# Autodesk Inventor assembly: Camera stage V2 assembly
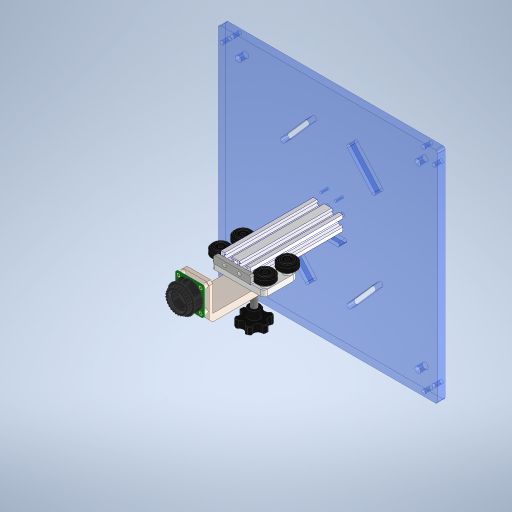
[picture p0: Inventor's stored thumbnail of the model, 512x512]
Saved by Autodesk Inventor 2023 (Build 270158000, 158)
## iProperties
Created: 2020-12-15
Part Number: Camera stage V2 assembly
Document SubType Name: Assembly
Designer: ferrerx
Author: ferrerx
## Documents named in this file (12)
- C:\Users\ferrerx\Desktop\Projects\Prieto-Godino Lab\Drosophila Larvae Behavioural Device\Device design V4\Inventor Assembly\Camera stage V2\Camera stage V2 assembly.iam
- C:\Users\ferrerx\Desktop\Projects\Prieto-Godino Lab\Drosophila Larvae Behavioural Device\Device design V4\Inventor Assembly\cart_spacer.ipt
- C:\Users\ferrerx\Desktop\Projects\Prieto-Godino Lab\Drosophila Larvae Behavioural Device\Device design V4\Inventor Assembly\guide wheel.ipt
- C:\Users\ferrerx\Documents\Inventor\Content Center Files\R2020\en-US\AS 1427(10)\AS 1427 - M5 x 30(7).ipt
- C:\Users\ferrerx\Documents\Inventor\Content Center Files\R2020\en-US\BS 4183(1)\BS 4183 - M5(1).ipt
- C:\Users\ferrerx\Desktop\Projects\Prieto-Godino Lab\Drosophila Larvae Behavioural Device\Device design V4\Inventor Assembly\Camera stage V2\Camera_cart_V2.ipt
- C:\Users\ferrerx\Desktop\Projects\Prieto-Godino Lab\Drosophila Larvae Behavioural Device\Device design V4\Inventor Assembly\Camera stage V2\aluminum profile camera stage.ipt
- C:\Users\ferrerx\Desktop\Projects\Prieto-Godino Lab\Drosophila Larvae Behavioural Device\Device design V4\Inventor Assembly\Camera stage V2\RaspberryPi HQ Camera.ipt
- C:\Users\ferrerx\Desktop\Projects\Prieto-Godino Lab\Drosophila Larvae Behavioural Device\Device design V4\Inventor Assembly\Camera stage V2\Raspberry pi HQ camera holder V2.ipt
- C:\Users\ferrerx\Desktop\Projects\Prieto-Godino Lab\Drosophila Larvae Behavioural Device\Device design V4\Inventor Assembly\Camera stage V2\Z stage Roof V2.ipt
- C:\Users\ferrerx\Desktop\Projects\Prieto-Godino Lab\Drosophila Larvae Behavioural Device\Device design V4\Inventor Assembly\Camera stage V2\Thumb screw.ipt
- C:\Users\ferrerx\Desktop\Projects\Prieto-Godino Lab\Drosophila Larvae Behavioural Device\Device design V4\Inventor Assembly\Camera stage V2\Stop.ipt
## Components (23 placed, 11 different names)
1. cart_spacer:1 — Mate:16, Mate:47, Mate:48, Mate:51
2. cart_spacer:2 — Mate:18, Mate:49, Mate:50, Mate:53
3. cart_spacer:3 — Mate:19, Mate:43, Mate:54
4. cart_spacer:4 — Mate:17, Mate:45, Mate:46, Mate:52
5. guide wheel:1 — Mate:18, Mate:42, Mate:50
6. guide wheel:2 — Mate:17, Mate:40, Mate:46
7. guide wheel:3 — Mate:16, Mate:41, Mate:48
8. guide wheel:4 — Mate:19, Mate:39, Mate:44
9. AS 1427 (8) - Metric M5 x 30:1 — Mate:35
10. AS 1427 (8) - Metric M5 x 30:2 — Mate:36
11. AS 1427 (8) - Metric M5 x 30:3 — Mate:37
12. AS 1427 (8) - Metric M5 x 30:4 — Mate:38
13. BS 4183 - Metric M5:1 — Mate:36, Mate:41
14. BS 4183 - Metric M5:2 — Mate:35, Mate:40
15. BS 4183 - Metric M5:3 — Mate:38, Mate:42
16. BS 4183 - Metric M5:4 — Mate:37, Mate:39
17. Camera_cart_V2:1 — Mate:43, Mate:44, Mate:45, Mate:47, Mate:49, Mate:51, Mate:52, Mate:53, Mate:54, Mate:58, Mate:59, Mate:60, Mate:64
18. aluminum profile camera stage:1 — Mate:61, Mate:62, Mate:63, Mate:64, Flush:1, Mate:67, Mate:68, Mate:69, Mate:70
19. RaspberryPi HQ Camera:1 — Mate:55, Mate:56, Mate:57, Mate:66
20. Raspberry pi HQ camera holder V2:1 — Mate:55, Mate:56, Mate:57, Mate:58, Mate:59, Mate:60, Flush:1, Mate:65
21. Z stage Roof V2:1 — Mate:61, Mate:62, Mate:63
22. Thumb screw:1 — Mate:65
23. Stop:1 — Mate:68, Mate:69, Mate:70
## Relationships (41: Mate 40, Flush 1)
- Mate:16: cart_spacer:1 ↔ guide wheel:3
- Mate:17: cart_spacer:4 ↔ guide wheel:2
- Mate:18: cart_spacer:2 ↔ guide wheel:1
- Mate:19: cart_spacer:3 ↔ guide wheel:4
- Mate:35: AS 1427 (8) - Metric M5 x 30:1 ↔ BS 4183 - Metric M5:2
- Mate:36: AS 1427 (8) - Metric M5 x 30:2 ↔ BS 4183 - Metric M5:1
- Mate:37: AS 1427 (8) - Metric M5 x 30:3 ↔ BS 4183 - Metric M5:4
- Mate:38: AS 1427 (8) - Metric M5 x 30:4 ↔ BS 4183 - Metric M5:3
- Mate:39: guide wheel:4 ↔ BS 4183 - Metric M5:4
- Mate:40: guide wheel:2 ↔ BS 4183 - Metric M5:2
- Mate:41: guide wheel:3 ↔ BS 4183 - Metric M5:1
- Mate:42: guide wheel:1 ↔ BS 4183 - Metric M5:3
- Mate:43: cart_spacer:3 ↔ Camera_cart_V2:1
- Mate:44: guide wheel:4 ↔ Camera_cart_V2:1
- Mate:45: cart_spacer:4 ↔ Camera_cart_V2:1
- Mate:46: cart_spacer:4 ↔ guide wheel:2
- Mate:47: cart_spacer:1 ↔ Camera_cart_V2:1
- Mate:48: cart_spacer:1 ↔ guide wheel:3
- Mate:49: cart_spacer:2 ↔ Camera_cart_V2:1
- Mate:50: cart_spacer:2 ↔ guide wheel:1
- Mate:51: cart_spacer:1 ↔ Camera_cart_V2:1
- Mate:52: cart_spacer:4 ↔ Camera_cart_V2:1
- Mate:53: cart_spacer:2 ↔ Camera_cart_V2:1
- Mate:54: cart_spacer:3 ↔ Camera_cart_V2:1
- Mate:55: RaspberryPi HQ Camera:1 ↔ Raspberry pi HQ camera holder V2:1
- Mate:56: RaspberryPi HQ Camera:1 ↔ Raspberry pi HQ camera holder V2:1
- Mate:57: RaspberryPi HQ Camera:1 ↔ Raspberry pi HQ camera holder V2:1
- Mate:58: Camera_cart_V2:1 ↔ Raspberry pi HQ camera holder V2:1
- Mate:59: Camera_cart_V2:1 ↔ Raspberry pi HQ camera holder V2:1
- Mate:60: Camera_cart_V2:1 ↔ Raspberry pi HQ camera holder V2:1
- Mate:61: aluminum profile camera stage:1 ↔ Z stage Roof V2:1
- Mate:62: aluminum profile camera stage:1 ↔ Z stage Roof V2:1
- Mate:63: aluminum profile camera stage:1 ↔ Z stage Roof V2:1
- Mate:64 (1 mm): Camera_cart_V2:1 ↔ aluminum profile camera stage:1
- Flush:1 (1 mm): aluminum profile camera stage:1 ↔ Raspberry pi HQ camera holder V2:1
- Mate:65: Raspberry pi HQ camera holder V2:1 ↔ Thumb screw:1
- Mate:66: RaspberryPi HQ Camera:1
- Mate:67: aluminum profile camera stage:1
- Mate:68: aluminum profile camera stage:1 ↔ Stop:1
- Mate:69: aluminum profile camera stage:1 ↔ Stop:1
- Mate:70: aluminum profile camera stage:1 ↔ Stop:1
